# Autodesk Inventor assembly: IC
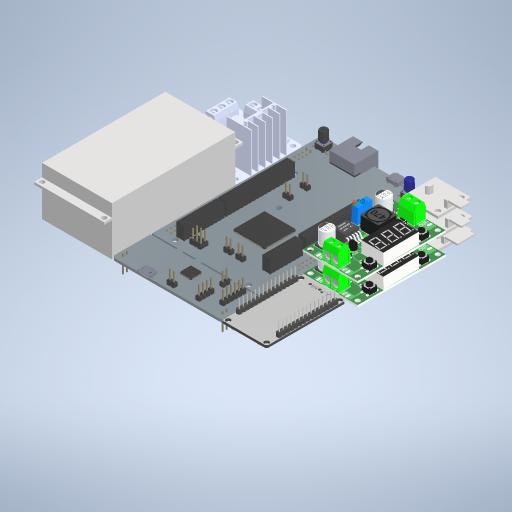
[picture p0: Inventor's stored thumbnail of the model, 512x512]
Saved by Autodesk Inventor 2024 (Build 280153000, 153)
## iProperties
Created: 2025-03-13
Part Number: IC
Document SubType Name: Assembly
Designer: 5454s
Author: 5454s
## Documents named in this file (10)
- C:\Users\5454s\OneDrive\桌面\Smart_fan\IC.iam
- C:\Users\5454s\OneDrive\桌面\Smart_fan\6.ESP-32_Predeterminado.ipt
- C:\Users\5454s\OneDrive\桌面\Smart_fan\NUCLEO-F429ZI--3DModel-STEP-56544.iam
- C:\Users\5454s\OneDrive\桌面\Smart_fan\DS18B20.ipt
- C:\Users\5454s\OneDrive\桌面\Smart_fan\IR_Receiver.ipt
- C:\Users\5454s\OneDrive\桌面\Smart_fan\L298N Driver.iam
- C:\Users\5454s\OneDrive\桌面\Smart_fan\LM2596_Modelo_3D.ipt
- C:\Users\5454s\OneDrive\桌面\Smart_fan\RTC.ipt
- C:\Users\5454s\OneDrive\桌面\Smart_fan\battery.ipt
- C:\Users\5454s\OneDrive\桌面\Smart_fan\SG90_v7.ipt
## Components (10 placed, 9 different names)
1. 6.ESP-32_Predeterminado:1 — Mate:66, Mate:67, Mate:71
2. NUCLEO-F429ZI--3DModel-STEP-56544:1 [sub-assembly] — Mate:17, Mate:19, Mate:43, Mate:44, Mate:51, Mate:52, Mate:54, Mate:55, Mate:63, Mate:64, Mate:66, Mate:67, Mate:68, Mate:70
3. DS18B20:1 — Mate:57, Mate:58
4. IR_Receiver:1 — Mate:2, Mate:3, Mate:4, Mate:57, Mate:58
5. L298N Driver:1 [sub-assembly] — Mate:62, Mate:63, Mate:70
6. LM2596_Modelo_3D:1 — Mate:5, Mate:6, Mate:7
7. LM2596_Modelo_3D:2 — Mate:5, Mate:6, Mate:7, Mate:51, Mate:52, Mate:56, Mate:71
8. RTC:1 — Mate:2, Mate:3, Mate:4, Mate:54, Mate:55, Mate:56
9. battery:1 — Mate:43, Mate:44, Mate:62, Mate:64, Mate:69
10. SG90_v7:1 — Mate:17, Mate:19
## Relationships (26: Mate 26)
- Mate:2: IR_Receiver:1 ↔ RTC:1
- Mate:3: IR_Receiver:1 ↔ RTC:1
- Mate:4 (6 mm): IR_Receiver:1 ↔ RTC:1
- Mate:5: LM2596_Modelo_3D:1 ↔ LM2596_Modelo_3D:2
- Mate:6 (12 mm): LM2596_Modelo_3D:1 ↔ LM2596_Modelo_3D:2
- Mate:7: LM2596_Modelo_3D:1 ↔ LM2596_Modelo_3D:2
- Mate:17: NUCLEO-F429ZI--3DModel-STEP-56544:1 ↔ SG90_v7:1
- Mate:19 (1 mm): NUCLEO-F429ZI--3DModel-STEP-56544:1 ↔ SG90_v7:1
- Mate:43: NUCLEO-F429ZI--3DModel-STEP-56544:1 ↔ battery:1
- Mate:44: NUCLEO-F429ZI--3DModel-STEP-56544:1 ↔ battery:1
- Mate:51: NUCLEO-F429ZI--3DModel-STEP-56544:1 ↔ LM2596_Modelo_3D:2
- Mate:52: NUCLEO-F429ZI--3DModel-STEP-56544:1 ↔ LM2596_Modelo_3D:2
- Mate:54: NUCLEO-F429ZI--3DModel-STEP-56544:1 ↔ RTC:1
- Mate:55: NUCLEO-F429ZI--3DModel-STEP-56544:1 ↔ RTC:1
- Mate:56: LM2596_Modelo_3D:2 ↔ RTC:1
- Mate:57 (9 mm): DS18B20:1 ↔ IR_Receiver:1
- Mate:58: DS18B20:1 ↔ IR_Receiver:1
- Mate:62: L298N Driver:1 ↔ battery:1
- Mate:63: NUCLEO-F429ZI--3DModel-STEP-56544:1 ↔ L298N Driver:1
- Mate:64: NUCLEO-F429ZI--3DModel-STEP-56544:1 ↔ battery:1
- Mate:66: 6.ESP-32_Predeterminado:1 ↔ NUCLEO-F429ZI--3DModel-STEP-56544:1
- Mate:67: 6.ESP-32_Predeterminado:1 ↔ NUCLEO-F429ZI--3DModel-STEP-56544:1
- Mate:68: NUCLEO-F429ZI--3DModel-STEP-56544:1
- Mate:69: battery:1
- Mate:70: NUCLEO-F429ZI--3DModel-STEP-56544:1 ↔ L298N Driver:1
- Mate:71 (1 mm): 6.ESP-32_Predeterminado:1 ↔ LM2596_Modelo_3D:2
